# Autodesk Inventor assembly: Assembly1.1
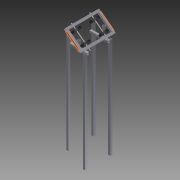
[picture p0: Inventor's stored thumbnail of the model, 180x180]
Saved by Autodesk Inventor 2011 SP1 (Build 150282100, 282)
## iProperties
Created: 2012-01-14
Part Number: Assembly1.1
Document SubType Name: Assembly
Designer: Christopher
Author: Christopher
## Documents named in this file (8)
- C:\Users\Christopher\Documents\Christopher\FIRST\Inventor files\2012\4 wheel kicker version 1\Assembly1.1.iam
- C:\Users\Christopher\Documents\Christopher\FIRST\Inventor files\2012\4 wheel kicker version 1\9 in .125 aluminum tube.ipt
- C:\Users\Christopher\Documents\Christopher\FIRST\Inventor files\2012\4 wheel kicker version 1\18 inch tube.ipt
- C:\Users\Christopher\Documents\Christopher\FIRST\Inventor files\2012\4 wheel kicker version 1\wheel.ipt
- C:\Users\Christopher\Documents\Christopher\FIRST\Inventor files\2012\4 wheel kicker version 1\axle1 .5inch.ipt
- C:\Users\Christopher\Documents\Christopher\FIRST\Inventor files\2012\tower first design\towerfrontdraft.ipt
- C:\Users\Christopher\Documents\Christopher\FIRST\Inventor files\2012\tower first design\towerbracebackwards.ipt
- C:\Users\Christopher\Documents\Christopher\FIRST\Inventor files\2012\tower first design\short thing.ipt
## Components (18 placed, 7 different names)
1. 18 inch tube:2 — Insert:1, Insert:2, Mate:1, Flush:1, Flush:2, Flush:3, Mate:6, Flush:12
2. wheel:1 — Insert:3
3. wheel:2 — Insert:4
4. wheel:3 — Insert:9
5. wheel:4 — Insert:10
6. axle1 .5inch:1 — Insert:1, Insert:3, Insert:9
7. axle1 .5inch:2 — Insert:2, Insert:4, Insert:10
8. 9 in .125 aluminum tube:1 — Mate:1, Flush:1, Flush:2, Mate:17, Flush:27, Flush:28
9. 9 in .125 aluminum tube:2 — Flush:3, Mate:6, Flush:12
10. towerfrontdraft:1 — Mate:10, Flush:19, Flush:20, Mate:18
11. towerfrontdraft:2 — Mate:9, Flush:17, Flush:18, Mate:14
12. towerbracebackwards:1 — Mate:10, Flush:19, Flush:20, Mate:12, Flush:23, Flush:24, Mate:15, Flush:26
13. towerbracebackwards:2 — Mate:9, Flush:17, Flush:18, Mate:11, Flush:21, Flush:22, Mate:13, Flush:25
14. towerfrontdraft:3 — Mate:11, Flush:21, Flush:22
15. towerfrontdraft:4 — Mate:12, Flush:23, Flush:24
16. short thing:1 — Mate:13, Flush:25, Mate:14
17. short thing:2 — Mate:15, Flush:26, Mate:18
18. 18 inch tube:3 — Mate:17, Flush:27, Flush:28
## Relationships (33: Flush 16, Mate 11, Insert 6)
- Insert:1 (-12.7 mm): 18 inch tube:2 ↔ axle1 .5inch:1
- Insert:2 (-12.7 mm): 18 inch tube:2 ↔ axle1 .5inch:2
- Insert:3 (66.04 mm): wheel:1 ↔ axle1 .5inch:1
- Insert:4 (66.04 mm): wheel:2 ↔ axle1 .5inch:2
- Mate:1: 18 inch tube:2 ↔ 9 in .125 aluminum tube:1
- Flush:1: 18 inch tube:2 ↔ 9 in .125 aluminum tube:1
- Flush:2: 18 inch tube:2 ↔ 9 in .125 aluminum tube:1
- Insert:9 (205.74 mm): wheel:3 ↔ axle1 .5inch:1
- Insert:10 (205.74 mm): wheel:4 ↔ axle1 .5inch:2
- Flush:3: 18 inch tube:2 ↔ 9 in .125 aluminum tube:2
- Mate:6: 18 inch tube:2 ↔ 9 in .125 aluminum tube:2
- Flush:12: 18 inch tube:2 ↔ 9 in .125 aluminum tube:2
- Mate:9: towerfrontdraft:2 ↔ towerbracebackwards:2
- Flush:17: towerfrontdraft:2 ↔ towerbracebackwards:2
- Flush:18: towerfrontdraft:2 ↔ towerbracebackwards:2
- Mate:10: towerfrontdraft:1 ↔ towerbracebackwards:1
- Flush:19: towerfrontdraft:1 ↔ towerbracebackwards:1
- Flush:20: towerfrontdraft:1 ↔ towerbracebackwards:1
- Mate:11: towerbracebackwards:2 ↔ towerfrontdraft:3
- Flush:21: towerbracebackwards:2 ↔ towerfrontdraft:3
- Flush:22 (101.6 mm): towerbracebackwards:2 ↔ towerfrontdraft:3
- Mate:12: towerbracebackwards:1 ↔ towerfrontdraft:4
- Flush:23: towerbracebackwards:1 ↔ towerfrontdraft:4
- Flush:24 (101.6 mm): towerbracebackwards:1 ↔ towerfrontdraft:4
- Mate:13: towerbracebackwards:2 ↔ short thing:1
- Flush:25: towerbracebackwards:2 ↔ short thing:1
- Mate:14 (50.8 mm): towerfrontdraft:2 ↔ short thing:1
- Mate:15: towerbracebackwards:1 ↔ short thing:2
- Flush:26: towerbracebackwards:1 ↔ short thing:2
- Mate:17: 9 in .125 aluminum tube:1 ↔ 18 inch tube:3
- Flush:27: 9 in .125 aluminum tube:1 ↔ 18 inch tube:3
- Flush:28: 9 in .125 aluminum tube:1 ↔ 18 inch tube:3
- Mate:18 (50.8 mm): towerfrontdraft:1 ↔ short thing:2
